# Autodesk Inventor assembly: Mark1o
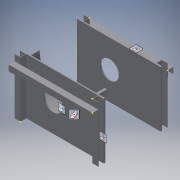
[picture p0: Inventor's stored thumbnail of the model, 180x180]
Saved by Autodesk Inventor 2017 (Build 210142000, 142)
## iProperties
Created: 2016-09-18
Part Number: Mark1o
Document SubType Name: Assembly
Designer: Spartacles
Author: Spartacles
## Documents named in this file (5)
- C:\Users\Spartacles\Desktop\FTC Parts\2016launcher\Mark1o.iam
- C:\Users\Spartacles\Desktop\FTC Parts\2016launcher\BallPath\BallPath180.ipt
- C:\Users\Spartacles\Desktop\FTC Parts\2016launcher\ShooterWall\ShooterWall2.ipt
- C:\Users\Spartacles\Desktop\FTC Parts\2016launcher\BeamSolid18\BeamSolid18.ipt
- C:\Users\Spartacles\Desktop\FTC Parts\2016launcher\BeamSolid18\BeamSolid14.ipt
## Components (9 placed, 4 different names)
1. BallPath180:1 — Mate:6, Mate:8, Flush:9
2. ShooterWall2:1 — Mate:10, Flush:12, Flush:13, Mate:11, Flush:14, Flush:15
3. ShooterWall2:2 — Mate:1, Flush:3, Flush:4, Mate:3, Flush:5, Flush:6, Mate:6, Mate:8, Flush:9
4. BeamSolid18:2 — Mate:5, Flush:10, Flush:11, Mate:9
5. BeamSolid18:3 — Flush:16, Flush:17, Mate:12
6. BeamSolid14:1 — Mate:10, Flush:12, Flush:13, Flush:17, Mate:12
7. BeamSolid14:2 — Mate:3, Flush:5, Flush:6, Flush:10, Flush:11
8. BeamSolid14:3 — Mate:11, Flush:14, Flush:15, Flush:16
9. BeamSolid14:4 — Mate:1, Flush:3, Flush:4, Mate:5, Mate:9
## Relationships (22: Flush 13, Mate 9)
- Mate:1: ShooterWall2:2 ↔ BeamSolid14:4
- Flush:3: ShooterWall2:2 ↔ BeamSolid14:4
- Flush:4: ShooterWall2:2 ↔ BeamSolid14:4
- Mate:3: ShooterWall2:2 ↔ BeamSolid14:2
- Flush:5: ShooterWall2:2 ↔ BeamSolid14:2
- Flush:6: ShooterWall2:2 ↔ BeamSolid14:2
- Mate:5: BeamSolid18:2 ↔ BeamSolid14:4
- Mate:6: BallPath180:1 ↔ ShooterWall2:2
- Mate:8: BallPath180:1 ↔ ShooterWall2:2
- Flush:9 (50.8 mm): BallPath180:1 ↔ ShooterWall2:2
- Flush:10 (34.798 mm): BeamSolid18:2 ↔ BeamSolid14:2
- Flush:11: BeamSolid18:2 ↔ BeamSolid14:2
- Mate:9: BeamSolid18:2 ↔ BeamSolid14:4
- Mate:10: ShooterWall2:1 ↔ BeamSolid14:1
- Flush:12: ShooterWall2:1 ↔ BeamSolid14:1
- Flush:13: ShooterWall2:1 ↔ BeamSolid14:1
- Mate:11: ShooterWall2:1 ↔ BeamSolid14:3
- Flush:14: ShooterWall2:1 ↔ BeamSolid14:3
- Flush:15: ShooterWall2:1 ↔ BeamSolid14:3
- Flush:16 (34.798 mm): BeamSolid18:3 ↔ BeamSolid14:3
- Flush:17: BeamSolid18:3 ↔ BeamSolid14:1
- Mate:12: BeamSolid18:3 ↔ BeamSolid14:1
